# Autodesk Inventor assembly: Console Assembly
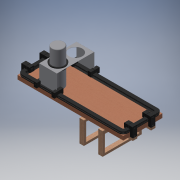
[picture p0: Inventor's stored thumbnail of the model, 180x180]
Saved by Autodesk Inventor 2019 (Build 230136000, 136)
## iProperties
Created: 2020-12-25
Part Number: Console Assembly
Document SubType Name: Assembly
Designer: John
Author: John
## Documents named in this file (16)
- C:\Users\John\Desktop\Truck Console Project\Console Assembly.iam
- C:\Users\John\Desktop\Truck Console Project\Deck.ipt
- C:\Users\John\Desktop\Truck Console Project\Rail Segment.ipt
- C:\Users\John\Desktop\Truck Console Project\Rail Corner 2.ipt
- C:\Users\John\Desktop\Truck Console Project\92196A197_18-8 STAINLESS STEEL SOCKET HEAD SCREW.ipt
- C:\Users\John\Desktop\Truck Console Project\94831A005_LOW-STRENGTH STEEL SERRATED-FLANGE LOCKNUT.ipt
- C:\Users\John\Desktop\Truck Console Project\Rail Corner.ipt
- C:\Users\John\Desktop\Truck Console Project\Corner Clamp.ipt
- C:\Users\John\Desktop\Truck Console Project\Cup Holder Bracket Mirror.ipt
- C:\Users\John\Desktop\Truck Console Project\Cup Holder Bracket.ipt
- C:\Users\John\Desktop\Truck Console Project\Cup Holder Sheet Metal.ipt
- C:\Users\John\Desktop\Truck Console Project\Water Bottle Ring.ipt
- C:\Users\John\Desktop\Truck Console Project\Water Bottle Model.ipt
- C:\Users\John\Desktop\Truck Console Project\1x2 Horizontal.ipt
- C:\Users\John\Desktop\Truck Console Project\1x2 Longitudinal.ipt
- C:\Users\John\Desktop\Truck Console Project\1x2 Risers.ipt
## Components (38 placed, 15 different names)
1. Deck:1 — Mate:32, Flush:1, Mate:33, Flush:2, Mate:35, Flush:3, Mate:36, Mate:38, Flush:6, Flush:7, Mate:40, Flush:9, Mate:41, Flush:10, Mate:43, Flush:11, Mate:45, Mate:47, Mate:49, Mate:51, Flush:15, Mate:59, Flush:23, Flush:29, Mate:69, Mate:72, Flush:40, Flush:47
2. 92196A197_18-8 STAINLESS STEEL SOCKET HEAD SCREW:1 — Mate:30, Mate:31
3. 94831A005_LOW-STRENGTH STEEL SERRATED-FLANGE LOCKNUT:1
4. Corner Clamp:2 — Flush:22, Flush:33, Flush:34, Mate:64, Flush:38, Mate:71, Flush:39
5. Corner Clamp:3 — Mate:59, Flush:20, Flush:21, Flush:35
6. Corner Clamp:4 — Flush:20, Flush:21, Flush:22
7. Cup Holder Bracket Mirror:1 — Flush:28, Flush:29, Flush:30, Flush:32
8. Cup Holder Bracket Mirror:2 — Flush:23, Flush:24, Flush:25, Flush:26, Flush:27, Mate:60, Mate:62, Flush:31, Mate:65
9. Cup Holder Bracket:1 — Flush:27, Flush:30, Flush:31
10. Cup Holder Bracket:2 — Flush:25, Flush:26, Flush:28, Mate:61, Flush:32
11. Cup Holder Sheet Metal:1 — Mate:60, Mate:61, Mate:62, Mate:65, Mate:66, Mate:67
12. Corner Clamp:5 — Flush:33, Flush:34, Flush:35, Mate:70, Flush:36, Flush:37, Mate:81, Mate:82
13. Water Bottle Ring:1 — Mate:66, Mate:67, Mate:68
14. Water Bottle Model:1 — Mate:68, Mate:69
15. 1x2 Horizontal:1 — Mate:73, Flush:40, Mate:74, Flush:41, Flush:42, Mate:75, Flush:43, Flush:44
16. 1x2 Longitudinal:1 — Mate:70, Flush:36, Flush:37, Mate:73, Mate:77, Mate:83, Mate:84
17. 1x2 Longitudinal:2 — Flush:38, Mate:71, Flush:39, Mate:72
18. 1x2 Horizontal:2 — Mate:76, Flush:45, Flush:46
19. 1x2 Risers:1 — Mate:75, Flush:43, Flush:44, Mate:76, Flush:45, Flush:46
20. 1x2 Risers:2 — Mate:74, Flush:41, Flush:42
21. 1x2 Horizontal:3 — Mate:77, Flush:47, Mate:78, Flush:48, Flush:49, Mate:79, Flush:50, Flush:51
22. 1x2 Risers:3 — Mate:78, Flush:48, Flush:49, Mate:80, Flush:52, Flush:53
23. 1x2 Risers:4 — Mate:79, Flush:50, Flush:51
24. 1x2 Horizontal:4 — Mate:80, Flush:52, Flush:53
25. 94831A005_LOW-STRENGTH STEEL SERRATED-FLANGE LOCKNUT:2 — Mate:81, Mate:82
26. 92196A197_18-8 STAINLESS STEEL SOCKET HEAD SCREW:2 — Mate:83, Mate:84
27. Rail Segment:5 — Mate:30, Mate:31, Mate:32, Mate:34, Mate:39, Flush:8, Flush:9
28. Rail Corner 2:1 — Flush:2, Mate:35, Flush:3, Flush:5
29. Rail Corner:1 — Flush:1, Mate:33, Mate:34, Flush:4, Mate:37
30. Rail Segment:6 — Mate:36, Flush:4, Mate:37, Flush:5
31. Rail Corner 2:2 — Mate:38, Flush:6, Flush:7, Mate:44
32. Rail Segment:7 — Mate:39, Mate:40, Flush:8, Mate:42, Flush:24
33. Rail Segment:8 — Mate:41, Mate:42, Flush:10
34. Rail Segment:9 — Mate:43, Flush:11, Mate:44, Mate:46, Flush:12, Mate:64
35. Rail Corner:2 — Mate:45, Mate:46, Flush:12, Flush:13, Mate:48
36. Rail Segment:10 — Mate:47, Flush:13, Mate:48, Flush:14, Mate:50
37. Rail Segment:11 — Mate:49, Flush:14, Mate:50, Mate:52
38. Rail Segment:12 — Mate:51, Flush:15, Mate:52
## Relationships (97: Flush 49, Mate 48)
- Mate:30: 92196A197_18-8 STAINLESS STEEL SOCKET HEAD SCREW:1 ↔ Rail Segment:5
- Mate:31: 92196A197_18-8 STAINLESS STEEL SOCKET HEAD SCREW:1 ↔ Rail Segment:5
- Mate:32: Deck:1 ↔ Rail Segment:5
- Flush:1: Deck:1 ↔ Rail Corner:1
- Mate:33: Deck:1 ↔ Rail Corner:1
- Mate:34: Rail Segment:5 ↔ Rail Corner:1
- Flush:2: Deck:1 ↔ Rail Corner 2:1
- Mate:35: Deck:1 ↔ Rail Corner 2:1
- Flush:3: Deck:1 ↔ Rail Corner 2:1
- Mate:36: Deck:1 ↔ Rail Segment:6
- Flush:4: Rail Corner:1 ↔ Rail Segment:6
- Mate:37: Rail Corner:1 ↔ Rail Segment:6
- Flush:5: Rail Corner 2:1 ↔ Rail Segment:6
- Mate:38: Deck:1 ↔ Rail Corner 2:2
- Flush:6: Deck:1 ↔ Rail Corner 2:2
- Flush:7: Deck:1 ↔ Rail Corner 2:2
- Mate:39: Rail Segment:5 ↔ Rail Segment:7
- Mate:40: Deck:1 ↔ Rail Segment:7
- Flush:8: Rail Segment:5 ↔ Rail Segment:7
- Flush:9: Deck:1 ↔ Rail Segment:5
- Mate:41: Deck:1 ↔ Rail Segment:8
- Mate:42: Rail Segment:7 ↔ Rail Segment:8
- Flush:10: Deck:1 ↔ Rail Segment:8
- Mate:43: Deck:1 ↔ Rail Segment:9
- Flush:11: Deck:1 ↔ Rail Segment:9
- Mate:44: Rail Corner 2:2 ↔ Rail Segment:9
- Mate:45: Deck:1 ↔ Rail Corner:2
- Mate:46: Rail Segment:9 ↔ Rail Corner:2
- Flush:12: Rail Segment:9 ↔ Rail Corner:2
- Mate:47: Deck:1 ↔ Rail Segment:10
- Flush:13: Rail Corner:2 ↔ Rail Segment:10
- Mate:48: Rail Corner:2 ↔ Rail Segment:10
- Mate:49: Deck:1 ↔ Rail Segment:11
- Flush:14: Rail Segment:10 ↔ Rail Segment:11
- Mate:50: Rail Segment:10 ↔ Rail Segment:11
- Mate:51: Deck:1 ↔ Rail Segment:12
- Flush:15: Deck:1 ↔ Rail Segment:12
- Mate:52: Rail Segment:11 ↔ Rail Segment:12
- Mate:59: Deck:1 ↔ Corner Clamp:3
- Flush:20: Corner Clamp:3 ↔ Corner Clamp:4
- Flush:21: Corner Clamp:3 ↔ Corner Clamp:4
- Flush:22: Corner Clamp:2 ↔ Corner Clamp:4
- Flush:23 (-25.4889 mm): Deck:1 ↔ Cup Holder Bracket Mirror:2
- Flush:24 (26.2636 mm): Cup Holder Bracket Mirror:2 ↔ Rail Segment:7
- Flush:25: Cup Holder Bracket Mirror:2 ↔ Cup Holder Bracket:2
- Flush:26: Cup Holder Bracket Mirror:2 ↔ Cup Holder Bracket:2
- Flush:27: Cup Holder Bracket Mirror:2 ↔ Cup Holder Bracket:1
- Flush:28: Cup Holder Bracket Mirror:1 ↔ Cup Holder Bracket:2
- Flush:29 (-26.2636 mm): Deck:1 ↔ Cup Holder Bracket Mirror:1
- Flush:30: Cup Holder Bracket Mirror:1 ↔ Cup Holder Bracket:1
- Mate:60: Cup Holder Bracket Mirror:2 ↔ Cup Holder Sheet Metal:1
- Mate:61: Cup Holder Bracket:2 ↔ Cup Holder Sheet Metal:1
- Mate:62: Cup Holder Bracket Mirror:2 ↔ Cup Holder Sheet Metal:1
- Flush:31: Cup Holder Bracket Mirror:2 ↔ Cup Holder Bracket:1
- Flush:32: Cup Holder Bracket Mirror:1 ↔ Cup Holder Bracket:2
- Flush:33: Corner Clamp:2 ↔ Corner Clamp:5
- Flush:34: Corner Clamp:2 ↔ Corner Clamp:5
- Flush:35: Corner Clamp:3 ↔ Corner Clamp:5
- Mate:64 (0.635 mm): Corner Clamp:2 ↔ Rail Segment:9
- Mate:65: Cup Holder Bracket Mirror:2 ↔ Cup Holder Sheet Metal:1
- Mate:66: Cup Holder Sheet Metal:1 ↔ Water Bottle Ring:1
- Mate:67: Cup Holder Sheet Metal:1 ↔ Water Bottle Ring:1
- Mate:68: Water Bottle Ring:1 ↔ Water Bottle Model:1
- Mate:69: Deck:1 ↔ Water Bottle Model:1
- Mate:70: Corner Clamp:5 ↔ 1x2 Longitudinal:1
- Flush:36: Corner Clamp:5 ↔ 1x2 Longitudinal:1
- Flush:37: Corner Clamp:5 ↔ 1x2 Longitudinal:1
- Flush:38: Corner Clamp:2 ↔ 1x2 Longitudinal:2
- Mate:71: Corner Clamp:2 ↔ 1x2 Longitudinal:2
- Flush:39: Corner Clamp:2 ↔ 1x2 Longitudinal:2
- Mate:72: Deck:1 ↔ 1x2 Longitudinal:2
- Mate:73: 1x2 Horizontal:1 ↔ 1x2 Longitudinal:1
- Flush:40: Deck:1 ↔ 1x2 Horizontal:1
- Mate:74: 1x2 Horizontal:1 ↔ 1x2 Risers:2
- Flush:41: 1x2 Horizontal:1 ↔ 1x2 Risers:2
- Flush:42: 1x2 Horizontal:1 ↔ 1x2 Risers:2
- Mate:75: 1x2 Horizontal:1 ↔ 1x2 Risers:1
- Flush:43: 1x2 Horizontal:1 ↔ 1x2 Risers:1
- Flush:44: 1x2 Horizontal:1 ↔ 1x2 Risers:1
- Mate:76: 1x2 Horizontal:2 ↔ 1x2 Risers:1
- Flush:45: 1x2 Horizontal:2 ↔ 1x2 Risers:1
- Flush:46: 1x2 Horizontal:2 ↔ 1x2 Risers:1
- Mate:77: 1x2 Longitudinal:1 ↔ 1x2 Horizontal:3
- Flush:47: Deck:1 ↔ 1x2 Horizontal:3
- Mate:78: 1x2 Horizontal:3 ↔ 1x2 Risers:3
- Flush:48: 1x2 Horizontal:3 ↔ 1x2 Risers:3
- Flush:49: 1x2 Horizontal:3 ↔ 1x2 Risers:3
- Mate:79: 1x2 Horizontal:3 ↔ 1x2 Risers:4
- Flush:50: 1x2 Horizontal:3 ↔ 1x2 Risers:4
- Flush:51: 1x2 Horizontal:3 ↔ 1x2 Risers:4
- Mate:80: 1x2 Risers:3 ↔ 1x2 Horizontal:4
- Flush:52: 1x2 Risers:3 ↔ 1x2 Horizontal:4
- Flush:53: 1x2 Risers:3 ↔ 1x2 Horizontal:4
- Mate:81: Corner Clamp:5 ↔ 94831A005_LOW-STRENGTH STEEL SERRATED-FLANGE LOCKNUT:2
- Mate:82: Corner Clamp:5 ↔ 94831A005_LOW-STRENGTH STEEL SERRATED-FLANGE LOCKNUT:2
- Mate:83: 1x2 Longitudinal:1 ↔ 92196A197_18-8 STAINLESS STEEL SOCKET HEAD SCREW:2
- Mate:84: 1x2 Longitudinal:1 ↔ 92196A197_18-8 STAINLESS STEEL SOCKET HEAD SCREW:2
